# Autodesk Inventor assembly: buggy-assembly-group2
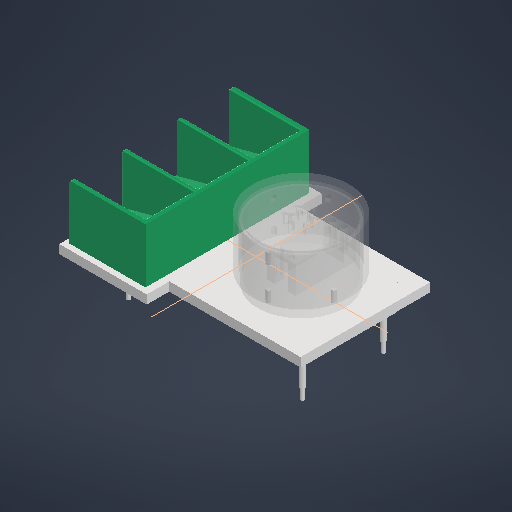
[picture p0: Inventor's stored thumbnail of the model, 512x512]
Saved by Autodesk Inventor 2026.2 (Build 302298010, 298A)
## iProperties
Created: 2026-02-23
Part Number: buggy-assembly-group2
Document SubType Name: Assembly
Designer: ts2104
Author: ts2104
## Documents named in this file (4)
- C:\Users\bobmi\OneDrive - Heriot-Watt University\Github\System-Project-G2\mechanical\buggy-assembly-group2.iam
- C:\Users\bobmi\OneDrive - Heriot-Watt University\Github\System-Project-G2\mechanical\rubbish-container-group2.ipt
- C:\Users\bobmi\OneDrive - Heriot-Watt University\Github\System-Project-G2\mechanical\crane-base-assembly.iam
- C:\Users\bobmi\OneDrive - Heriot-Watt University\Github\System-Project-G2\mechanical\Buggy_Body_assembly_ready.ipt
## Components (3 placed, 3 different names)
1. rubbish-container-group2:1 — Flush:1, Mate:4
2. crane-base-assembly:1 [sub-assembly] — Mate:5, Mate:6
3. Buggy_Body_assembly_ready:1 — Mate:1, Mate:2, Mate:3, Mate:4, Mate:5
## Relationships (7: Mate 6, Flush 1)
- Mate:1: Buggy_Body_assembly_ready:1
- Mate:2: Buggy_Body_assembly_ready:1
- Mate:3: Buggy_Body_assembly_ready:1
- Flush:1: rubbish-container-group2:1
- Mate:4: rubbish-container-group2:1 ↔ Buggy_Body_assembly_ready:1
- Mate:5: crane-base-assembly:1 ↔ Buggy_Body_assembly_ready:1
- Mate:6: crane-base-assembly:1
